# Autodesk Inventor assembly: TestBoxAssembly
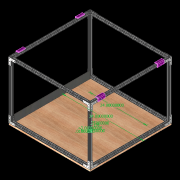
[picture p0: Inventor's stored thumbnail of the model, 180x180]
Saved by Autodesk Inventor 2022 (Build 260153000, 153)
## iProperties
Created: 2022-03-01
Part Number: TestBoxAssembly
Document SubType Name: Assembly
Designer: tandu
ScrewDiameter: 0.188 in
Author: tandu
## Documents named in this file (10)
- C:\Users\tandu\Documents\GrabCAD\Test Box\TestBoxAssembly.iam
- C:\Users\tandu\Documents\GrabCAD\Test Box\Floor.ipt
- C:\Users\tandu\Documents\GrabCAD\Test Box\Upright Extrusion 1010-24-CL.ipt
- C:\Users\tandu\Documents\GrabCAD\Test Box\Horizontal Extrusion 1010-32-CL.ipt
- C:\Users\tandu\Documents\GrabCAD\Test Box\DropInNuts 14162_m.ipt
- C:\Users\tandu\Documents\GrabCAD\Test Box\ConnectingPlatee.ipt
- C:\Users\tandu\Documents\GrabCAD\Test Box\Parameters.ipt
- C:\Users\tandu\Documents\GrabCAD\Test Box\10 32 0375 Screw 3042.ipt
- C:\Users\tandu\Documents\GrabCAD\Test Box\TopBracket.ipt
- C:\Users\tandu\Documents\GrabCAD\Test Box\KickPlate.ipt
## Components (43 placed, 9 different names)
1. Floor:1 — Mate:1, Flush:1, Flush:2, Mate:2, Mate:3, Mate:4, Flush:3, Flush:4, Flush:5, Flush:6, Flush:7, Flush:8, Mate:5, Mate:6, Mate:7, Mate:8, Flush:9, Flush:10, Flush:11, Flush:12, Flush:28, Flush:29, Mate:83
2. Parameters:1 — Flush:28, Flush:29
3. KickPlate:1 — Mate:82, Mate:83
4. Upright Extrusion 1010-24-CL:1 — Mate:1, Flush:1, Flush:2, Mate:9, Flush:15, Flush:16, Mate:14, Mate:74, Flush:45, Flush:61, Mate:51, Mate:68, Flush:71, Mate:75
5. Upright Extrusion 1010-24-CL:2 — Mate:4, Flush:5, Flush:6, Mate:11, Mate:16, Flush:20, Mate:80, Flush:32, Mate:44, Mate:64
6. Upright Extrusion 1010-24-CL:3 — Mate:3, Flush:3, Flush:4, Mate:10, Flush:17, Flush:18, Flush:19, Mate:15, Mate:46, Mate:63, Mate:61, Mate:66, Flush:59
7. Upright Extrusion 1010-24-CL:4 — Mate:2, Flush:7, Flush:8, Mate:12, Mate:13, Flush:13, Flush:14, Flush:23, Angle:1, Mate:17, Flush:25, Mate:18, Angle:2, Flush:27, Angle:3, Mate:21, Mate:76, Flush:36, Mate:73, Mate:58, Mate:81
8. Horizontal Extrusion 1010-32-CL:1 — Mate:5, Flush:10, Mate:10, Mate:45, Mate:47, Mate:62, Mate:82
9. Horizontal Extrusion 1010-32-CL:2 — Mate:8, Mate:9, Flush:9, Mate:49, Mate:67, Mate:50, Flush:62
10. Horizontal Extrusion 1010-32-CL:3 — Mate:7, Mate:12, Flush:12, Mate:39, Flush:42, Mate:40, Mate:69
11. Horizontal Extrusion 1010-32-CL:4 — Mate:6, Mate:11, Flush:11, Mate:24, Mate:78, Mate:25, Mate:77
12. Horizontal Extrusion 1010-32-CL:5 — Flush:15, Flush:16, Mate:14, Mate:48, Mate:65
13. Horizontal Extrusion 1010-32-CL:6 — Flush:17, Flush:18, Mate:15, Flush:70, Mate:54, Mate:55, Flush:66, Flush:67, Mate:59
14. Horizontal Extrusion 1010-32-CL:7 — Mate:13, Flush:13, Flush:14, Mate:26, Flush:37, Mate:41, Mate:70, Flush:47, Mate:42, Flush:48, Mate:52, Flush:65, Mate:71
15. Horizontal Extrusion 1010-32-CL:8 — Flush:19, Mate:16, Flush:20, Mate:19, Mate:23, Mate:79, Flush:69
16. DropInNuts 14162_m:3 — Angle:3, Mate:20, Mate:21
17. DropInNuts 14162_m:2 — Mate:18, Angle:2, Mate:22
18. DropInNuts 14162_m:1 — Flush:23, Angle:1, Mate:17, Flush:25, Mate:19
19. 10 32 0375 Screw 3042:1 — Insert:1
20. 10 32 0375 Screw 3042:2 — Insert:2
21. 10 32 0375 Screw 3042:3 — Insert:3
22. 10 32 0375 Screw 3042:4 — Insert:4
23. 10 32 0375 Screw 3042:5 — Insert:5
24. ConnectingPlatee:9 — Mate:45
25. ConnectingPlatee:10 — Mate:47, Mate:61, Mate:62
26. ConnectingPlatee:11 — Mate:46, Flush:70, Mate:63, Mate:56
27. ConnectingPlatee:12 — Mate:44, Mate:64, Mate:57, Mate:59
28. ConnectingPlatee:13 — Mate:48, Mate:65, Mate:66
29. ConnectingPlatee:14 — Mate:49, Flush:59, Mate:67
30. ConnectingPlatee:15 — Mate:50, Flush:61, Flush:62
31. ConnectingPlatee:16 — Mate:51, Flush:45, Mate:70
32. ConnectingPlatee:2 — Mate:41, Flush:71, Mate:71, Mate:72
33. ConnectingPlatee:3 — Mate:26, Flush:36, Flush:37, Mate:43
34. ConnectingPlatee:4 — Mate:39, Mate:73, Flush:42
35. ConnectingPlatee:5 — Mate:40, Mate:74, Mate:75, Mate:68, Mate:69
36. ConnectingPlatee:6 — Mate:25, Mate:76, Mate:77
37. ConnectingPlatee:7 — Mate:24, Flush:32, Mate:78
38. ConnectingPlatee:8 — Mate:23, Mate:79, Mate:80
39. ConnectingPlatee:1 — Flush:27, Mate:20, Mate:22, Insert:1, Insert:2, Insert:3, Insert:4, Insert:5, Mate:58, Mate:81, Flush:69
40. TopBracket:1 — Flush:47, Mate:42, Flush:48, Mate:43
41. TopBracket:2 — Mate:52, Flush:65, Mate:72
42. TopBracket:3 — Mate:55, Flush:66, Mate:57
43. TopBracket:4 — Mate:54, Flush:67, Mate:56
## Relationships (118: Mate 69, Flush 41, Insert 5, Angle 3)
- Mate:1: Floor:1 ↔ Upright Extrusion 1010-24-CL:1
- Flush:1: Floor:1 ↔ Upright Extrusion 1010-24-CL:1
- Flush:2: Floor:1 ↔ Upright Extrusion 1010-24-CL:1
- Mate:2: Floor:1 ↔ Upright Extrusion 1010-24-CL:4
- Mate:3: Floor:1 ↔ Upright Extrusion 1010-24-CL:3
- Mate:4: Floor:1 ↔ Upright Extrusion 1010-24-CL:2
- Flush:3: Floor:1 ↔ Upright Extrusion 1010-24-CL:3
- Flush:4: Floor:1 ↔ Upright Extrusion 1010-24-CL:3
- Flush:5: Floor:1 ↔ Upright Extrusion 1010-24-CL:2
- Flush:6: Floor:1 ↔ Upright Extrusion 1010-24-CL:2
- Flush:7: Floor:1 ↔ Upright Extrusion 1010-24-CL:4
- Flush:8: Floor:1 ↔ Upright Extrusion 1010-24-CL:4
- Mate:5: Floor:1 ↔ Horizontal Extrusion 1010-32-CL:1
- Mate:6: Floor:1 ↔ Horizontal Extrusion 1010-32-CL:4
- Mate:7: Floor:1 ↔ Horizontal Extrusion 1010-32-CL:3
- Mate:8: Floor:1 ↔ Horizontal Extrusion 1010-32-CL:2
- Mate:9: Upright Extrusion 1010-24-CL:1 ↔ Horizontal Extrusion 1010-32-CL:2
- Flush:9: Floor:1 ↔ Horizontal Extrusion 1010-32-CL:2
- Flush:10: Floor:1 ↔ Horizontal Extrusion 1010-32-CL:1
- Mate:10: Upright Extrusion 1010-24-CL:3 ↔ Horizontal Extrusion 1010-32-CL:1
- Mate:11: Upright Extrusion 1010-24-CL:2 ↔ Horizontal Extrusion 1010-32-CL:4
- Flush:11: Floor:1 ↔ Horizontal Extrusion 1010-32-CL:4
- Mate:12: Upright Extrusion 1010-24-CL:4 ↔ Horizontal Extrusion 1010-32-CL:3
- Flush:12: Floor:1 ↔ Horizontal Extrusion 1010-32-CL:3
- Mate:13: Upright Extrusion 1010-24-CL:4 ↔ Horizontal Extrusion 1010-32-CL:7
- Flush:13: Upright Extrusion 1010-24-CL:4 ↔ Horizontal Extrusion 1010-32-CL:7
- Flush:14: Upright Extrusion 1010-24-CL:4 ↔ Horizontal Extrusion 1010-32-CL:7
- Flush:15: Upright Extrusion 1010-24-CL:1 ↔ Horizontal Extrusion 1010-32-CL:5
- Flush:16: Upright Extrusion 1010-24-CL:1 ↔ Horizontal Extrusion 1010-32-CL:5
- Flush:17: Upright Extrusion 1010-24-CL:3 ↔ Horizontal Extrusion 1010-32-CL:6
- Flush:18: Upright Extrusion 1010-24-CL:3 ↔ Horizontal Extrusion 1010-32-CL:6
- Flush:19: Upright Extrusion 1010-24-CL:3 ↔ Horizontal Extrusion 1010-32-CL:8
- Mate:14: Upright Extrusion 1010-24-CL:1 ↔ Horizontal Extrusion 1010-32-CL:5
- Mate:15: Upright Extrusion 1010-24-CL:3 ↔ Horizontal Extrusion 1010-32-CL:6
- Mate:16: Upright Extrusion 1010-24-CL:2 ↔ Horizontal Extrusion 1010-32-CL:8
- Flush:20: Upright Extrusion 1010-24-CL:2 ↔ Horizontal Extrusion 1010-32-CL:8
- Flush:23: Upright Extrusion 1010-24-CL:4 ↔ DropInNuts 14162_m:1
- Angle:1 (180 deg): Upright Extrusion 1010-24-CL:4 ↔ DropInNuts 14162_m:1
- Mate:17: Upright Extrusion 1010-24-CL:4 ↔ DropInNuts 14162_m:1
- Flush:25: Upright Extrusion 1010-24-CL:4 ↔ DropInNuts 14162_m:1
- Mate:18: Upright Extrusion 1010-24-CL:4 ↔ DropInNuts 14162_m:2
- Angle:2 (180 deg): Upright Extrusion 1010-24-CL:4 ↔ DropInNuts 14162_m:2
- Mate:19: Horizontal Extrusion 1010-32-CL:8 ↔ DropInNuts 14162_m:1
- Flush:27: Upright Extrusion 1010-24-CL:4 ↔ ConnectingPlatee:1
- Flush:28: Floor:1 ↔ Parameters:1
- Flush:29: Floor:1 ↔ Parameters:1
- Angle:3 (0 deg): Upright Extrusion 1010-24-CL:4 ↔ DropInNuts 14162_m:3
- Mate:20: DropInNuts 14162_m:3 ↔ ConnectingPlatee:1
- Mate:21: Upright Extrusion 1010-24-CL:4 ↔ DropInNuts 14162_m:3
- Mate:22: DropInNuts 14162_m:2 ↔ ConnectingPlatee:1
- Insert:1: 10 32 0375 Screw 3042:1 ↔ ConnectingPlatee:1
- Insert:2: 10 32 0375 Screw 3042:2 ↔ ConnectingPlatee:1
- Insert:3: 10 32 0375 Screw 3042:3 ↔ ConnectingPlatee:1
- Insert:4: 10 32 0375 Screw 3042:4 ↔ ConnectingPlatee:1
- Insert:5: 10 32 0375 Screw 3042:5 ↔ ConnectingPlatee:1
- Mate:23: Horizontal Extrusion 1010-32-CL:8 ↔ ConnectingPlatee:8
- Mate:79: Horizontal Extrusion 1010-32-CL:8 ↔ ConnectingPlatee:8
- Mate:80: Upright Extrusion 1010-24-CL:2 ↔ ConnectingPlatee:8
- Mate:24: Horizontal Extrusion 1010-32-CL:4 ↔ ConnectingPlatee:7
- Flush:32: Upright Extrusion 1010-24-CL:2 ↔ ConnectingPlatee:7
- Mate:78: Horizontal Extrusion 1010-32-CL:4 ↔ ConnectingPlatee:7
- Mate:25: Horizontal Extrusion 1010-32-CL:4 ↔ ConnectingPlatee:6
- Mate:76: Upright Extrusion 1010-24-CL:4 ↔ ConnectingPlatee:6
- Mate:77: Horizontal Extrusion 1010-32-CL:4 ↔ ConnectingPlatee:6
- Mate:26: Horizontal Extrusion 1010-32-CL:7 ↔ ConnectingPlatee:3
- Flush:36: Upright Extrusion 1010-24-CL:4 ↔ ConnectingPlatee:3
- Flush:37: Horizontal Extrusion 1010-32-CL:7 ↔ ConnectingPlatee:3
- Mate:39: Horizontal Extrusion 1010-32-CL:3 ↔ ConnectingPlatee:4
- Mate:73: Upright Extrusion 1010-24-CL:4 ↔ ConnectingPlatee:4
- Flush:42: Horizontal Extrusion 1010-32-CL:3 ↔ ConnectingPlatee:4
- Mate:40: Horizontal Extrusion 1010-32-CL:3 ↔ ConnectingPlatee:5
- Mate:74: Upright Extrusion 1010-24-CL:1 ↔ ConnectingPlatee:5
- Mate:75: Upright Extrusion 1010-24-CL:1 ↔ ConnectingPlatee:5
- Mate:41: Horizontal Extrusion 1010-32-CL:7 ↔ ConnectingPlatee:2
- Flush:45: Upright Extrusion 1010-24-CL:1 ↔ ConnectingPlatee:16
- Mate:70: Horizontal Extrusion 1010-32-CL:7 ↔ ConnectingPlatee:16
- Flush:47: Horizontal Extrusion 1010-32-CL:7 ↔ TopBracket:1
- Mate:42: Horizontal Extrusion 1010-32-CL:7 ↔ TopBracket:1
- Flush:48: Horizontal Extrusion 1010-32-CL:7 ↔ TopBracket:1
- Mate:43 (3.175 mm): ConnectingPlatee:3 ↔ TopBracket:1
- Mate:44: Upright Extrusion 1010-24-CL:2 ↔ ConnectingPlatee:12
- Mate:64: Upright Extrusion 1010-24-CL:2 ↔ ConnectingPlatee:12
- Mate:45: Horizontal Extrusion 1010-32-CL:1 ↔ ConnectingPlatee:9
- Mate:59: Horizontal Extrusion 1010-32-CL:6 ↔ ConnectingPlatee:12
- Mate:46: Upright Extrusion 1010-24-CL:3 ↔ ConnectingPlatee:11
- Flush:70: Horizontal Extrusion 1010-32-CL:6 ↔ ConnectingPlatee:11
- Mate:63: Upright Extrusion 1010-24-CL:3 ↔ ConnectingPlatee:11
- Mate:47: Horizontal Extrusion 1010-32-CL:1 ↔ ConnectingPlatee:10
- Mate:61: Upright Extrusion 1010-24-CL:3 ↔ ConnectingPlatee:10
- Mate:62: Horizontal Extrusion 1010-32-CL:1 ↔ ConnectingPlatee:10
- Mate:48: Horizontal Extrusion 1010-32-CL:5 ↔ ConnectingPlatee:13
- Mate:65: Horizontal Extrusion 1010-32-CL:5 ↔ ConnectingPlatee:13
- Mate:66: Upright Extrusion 1010-24-CL:3 ↔ ConnectingPlatee:13
- Mate:49: Horizontal Extrusion 1010-32-CL:2 ↔ ConnectingPlatee:14
- Flush:59: Upright Extrusion 1010-24-CL:3 ↔ ConnectingPlatee:14
- Mate:67: Horizontal Extrusion 1010-32-CL:2 ↔ ConnectingPlatee:14
- Mate:50: Horizontal Extrusion 1010-32-CL:2 ↔ ConnectingPlatee:15
- Flush:61: Upright Extrusion 1010-24-CL:1 ↔ ConnectingPlatee:15
- Flush:62: Horizontal Extrusion 1010-32-CL:2 ↔ ConnectingPlatee:15
- Mate:51: Upright Extrusion 1010-24-CL:1 ↔ ConnectingPlatee:16
- Mate:68: Upright Extrusion 1010-24-CL:1 ↔ ConnectingPlatee:5
- Mate:69: Horizontal Extrusion 1010-32-CL:3 ↔ ConnectingPlatee:5
- Mate:52: Horizontal Extrusion 1010-32-CL:7 ↔ TopBracket:2
- Flush:65: Horizontal Extrusion 1010-32-CL:7 ↔ TopBracket:2
- Flush:71: Upright Extrusion 1010-24-CL:1 ↔ ConnectingPlatee:2
- Mate:54: Horizontal Extrusion 1010-32-CL:6 ↔ TopBracket:4
- Mate:55: Horizontal Extrusion 1010-32-CL:6 ↔ TopBracket:3
- Flush:66: Horizontal Extrusion 1010-32-CL:6 ↔ TopBracket:3
- Flush:67: Horizontal Extrusion 1010-32-CL:6 ↔ TopBracket:4
- Mate:56 (3.175 mm): ConnectingPlatee:11 ↔ TopBracket:4
- Mate:57 (3.175 mm): ConnectingPlatee:12 ↔ TopBracket:3
- Mate:58: Upright Extrusion 1010-24-CL:4 ↔ ConnectingPlatee:1
- Mate:81: Upright Extrusion 1010-24-CL:4 ↔ ConnectingPlatee:1
- Flush:69: Horizontal Extrusion 1010-32-CL:8 ↔ ConnectingPlatee:1
- Mate:71: Horizontal Extrusion 1010-32-CL:7 ↔ ConnectingPlatee:2
- Mate:72 (3.175 mm): ConnectingPlatee:2 ↔ TopBracket:2
- Mate:82: KickPlate:1 ↔ Horizontal Extrusion 1010-32-CL:1
- Mate:83: Floor:1 ↔ KickPlate:1
## Named parameters: ScrewDiameter = 4.7625 mm
